# Autodesk Inventor assembly: Screw jack Assembly
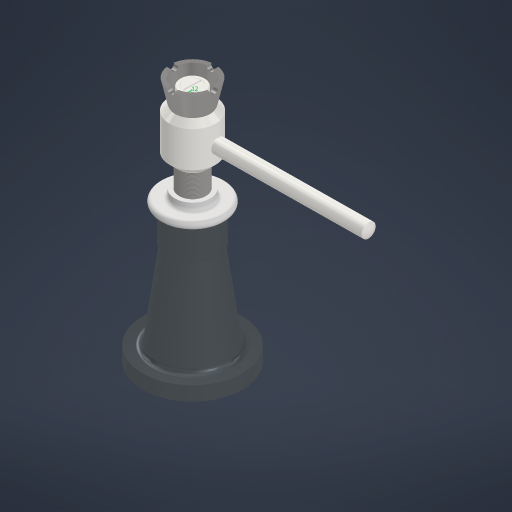
[picture p0: Inventor's stored thumbnail of the model, 512x512]
Saved by Autodesk Inventor 2023 (Build 270158000, 158)
## iProperties
Created: 2023-03-09
Part Number: Screw jack Assembly
Document SubType Name: Assembly
Designer: Kamraj S
Roll No.: 63
Author: Kamraj S
## Documents named in this file (8)
- C:\Users\kamra\OneDrive\Documents\Inventor\screw jack\screw jack Assembly.iam
- C:\Users\kamra\OneDrive\Documents\Inventor\screw jack\body.ipt
- C:\Users\kamra\OneDrive\Documents\Inventor\screw jack\nut.ipt
- C:\Users\kamra\OneDrive\Documents\Inventor\screw jack\screw.spindle.ipt
- C:\Users\kamra\OneDrive\Documents\Inventor\screw jack\cup.ipt
- C:\Users\kamra\OneDrive\Documents\Inventor\screw jack\washer.special.ipt
- C:\Users\kamra\OneDrive\Documents\Inventor\screw jack\tommybar.ipt
- C:\Users\kamra\OneDrive\Documents\Inventor\screw jack\csk.screw.ipt
## Components (7 placed, 7 different names)
1. body:1 — Insert:1
2. nut:1 — Insert:1, Cylindrical:1
3. screw.spindle:1 — Cylindrical:1, Insert:2, Rigid:1, Rigid:2, cskscrew
4. cup:1 — Insert:2
5. washer.special:1 — Rigid:1, cskscrew.1
6. csk.screw:1 — cskscrew, cskscrew.1
7. tommybar:1 — Rigid:2
## Relationships (7: Insert 2, WeldJoint 2, Mate 2, CylindricalJoint 1)
- Insert:1: body:1 ↔ nut:1
- Cylindrical:1: nut:1 ↔ screw.spindle:1
- Insert:2: screw.spindle:1 ↔ cup:1
- Rigid:1 [WeldJoint]: screw.spindle:1 ↔ washer.special:1
- Rigid:2 [WeldJoint]: screw.spindle:1 ↔ tommybar:1
- cskscrew [Mate]: screw.spindle:1 ↔ csk.screw:1
- cskscrew.1 [Mate]: washer.special:1 ↔ csk.screw:1
